# Autodesk Inventor assembly: CNC-YZ-axis- ASSEMBLY
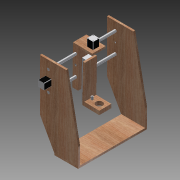
[picture p0: Inventor's stored thumbnail of the model, 180x180]
Saved by Autodesk Inventor 2015 (Build 190159000, 159)
## iProperties
Created: 2015-07-11
Part Number: CNC-YZ-axis- ASSEMBLY
Document SubType Name: Assembly
Designer: Bangladesh
Author: Bangladesh
## Documents named in this file (4)
- C:\Users\Alvi\Documents\CNC design files\CNC_1.0v\Assemblies\CNC-YZ-axis- ASSEMBLY.iam
- C:\Users\Alvi\Documents\CNC design files\CNC_1.0v\Assemblies\CNC-Y-axis- ASSEMBLY.iam
- C:\Users\Alvi\Documents\CNC design files\CNC_1.0v\Assemblies\CNC-Z-axis- ASSEMBLY.iam
- C:\Users\Alvi\Documents\CNC design files\CNC_1.0v\CNC-X-axis- moving platform.ipt
## Components (3 placed, 3 different names)
1. CNC-Y-axis- ASSEMBLY:1 [sub-assembly] — Mate:1, Mate:2, Mate:3, Mate:4
2. CNC-Z-axis- ASSEMBLY:1 [sub-assembly] — Mate:4
3. CNC-X-axis- moving platform:1 — Mate:1, Mate:2, Mate:3
## Relationships (4: Mate 4)
- Mate:1: CNC-Y-axis- ASSEMBLY:1 ↔ CNC-X-axis- moving platform:1
- Mate:2: CNC-Y-axis- ASSEMBLY:1 ↔ CNC-X-axis- moving platform:1
- Mate:3: CNC-Y-axis- ASSEMBLY:1 ↔ CNC-X-axis- moving platform:1
- Mate:4: CNC-Y-axis- ASSEMBLY:1 ↔ CNC-Z-axis- ASSEMBLY:1
